# Autodesk Inventor assembly: ChalkBot_MasterAssem
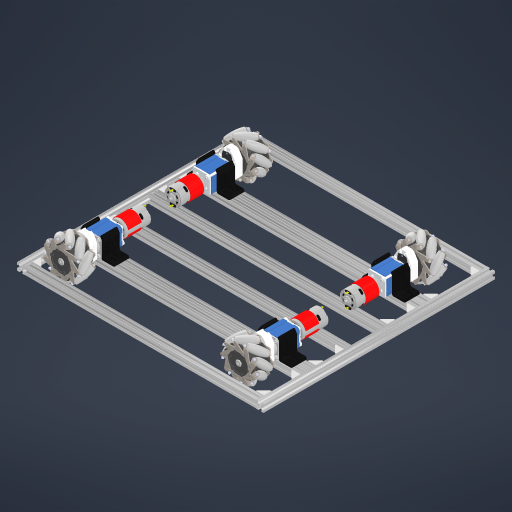
[picture p0: Inventor's stored thumbnail of the model, 512x512]
Saved by Autodesk Inventor 2024 (Build 280153000, 153)
## iProperties
Created: 2022-11-09
Part Number: ChalkBot_MasterAssem
Document SubType Name: Assembly
Designer: Dave
Author: Dave
## Documents named in this file (9)
- C:\Autodesk\ChalkBot Github\ChalkbotMechanical\Chalkbot1.0\ChalkBot_MasterAssem.iam
- C:\Users\Dave\Documents\GrabCAD\Chalk Bot\Chalkbot1.0\Chassis\V1\20x20 Channel.ipt
- C:\Autodesk\ChalkBot Github\ChalkbotMechanical\Chalkbot1.0\Chassis\V1\LeftMecanum-SubAssem01.iam
- C:\Autodesk\ChalkBot Github\ChalkbotMechanical\Chalkbot1.0\Chassis\V1\RightMecanum-SubAssem01.iam
- C:\Autodesk\ChalkBot Github\ChalkbotMechanical\Chalkbot1.0\Chassis\V1\20x20 90 Gusset.ipt
- C:\Autodesk\ChalkBot Github\ChalkbotMechanical\Chalkbot1.0\Chassis\V1\20x20 90 Gusset_MIR.ipt
- C:\Autodesk\ChalkBot Github\ChalkbotMechanical\Chalkbot1.0\Chassis\V1\20x20 90 Gusset_MIR1.ipt
- C:\Autodesk\ChalkBot Github\ChalkbotMechanical\Chalkbot1.0\Chassis\V1\20x20 90 Gusset_MIR_MIR.ipt
- C:\Autodesk\ChalkBot Github\ChalkbotMechanical\Chalkbot1.0\Chassis\V1\20x20 Channel\20x20 Channel-600.ipt
## Components (30 placed, 7 different names)
1. 20x20 Channel-600:1 — Flush:5, Flush:6, Flush:9, Flush:10, Mate:8, Flush:33, Mate:29, Tangent:7
2. 20x20 Channel-600:2 — Flush:6, Flush:7, Flush:8, Flush:9, Flush:27, Flush:28, Mate:4, Mate:5, Mate:6, Flush:32, Mate:28
3. 20x20 Channel-600:3 — Flush:7, Flush:8, Flush:15, Flush:16, Mate:12
4. 20x20 Channel-600:4 — Flush:2, Flush:3, Flush:12, Flush:13, Flush:17, Mate:16, Tangent:10
5. 20x20 Channel-600:5 — Flush:1, Flush:2, Flush:13, Flush:14, Mate:18, Tangent:9
6. 20x20 Channel-600:6 — Flush:1, Flush:14, Flush:29, Mate:20
7. 20x20 Channel-600:7 — Flush:3, Flush:4, Flush:11, Flush:12, Flush:16, Flush:17, Mate:15
8. 20x20 Channel-600:8 — Flush:4, Flush:5, Flush:10, Flush:11, Flush:15, Mate:11, Tangent:8
9. RightMecanum-SubAssem01:2 [sub-assembly] — Tangent:9, Tangent:10
10. LeftMecanum-SubAssem01:3 [sub-assembly]
11. RightMecanum-SubAssem01:1 [sub-assembly] — Flush:45
12. LeftMecanum-SubAssem01:4 [sub-assembly] — Tangent:7, Tangent:8, Flush:45
13. 20x20 Channel-600:9 — Flush:27, Flush:28, Mate:4, Flush:29, Flush:30, Flush:31, Mate:7, Mate:9, Flush:34, Mate:10, Mate:13, Flush:35, Mate:14, Mate:17, Mate:19, Mate:21
14. 20x20 Channel-600:10 — Flush:30, Flush:31, Mate:5, Mate:27, Flush:44
15. 20x20 90 Gusset:3 — Flush:34, Mate:10, Mate:11
16. 20x20 90 Gusset:4 — Mate:12, Mate:13, Flush:35, Flush:39
17. 20x20 90 Gusset:6 — Mate:6, Flush:32, Mate:7
18. 20x20 90 Gusset:7 — Mate:8, Mate:9, Flush:33
19. 20x20 90 Gusset_MIR:1 — Flush:36, Flush:37, Mate:16, Mate:17
20. 20x20 90 Gusset_MIR:2 — Flush:36, Flush:39, Mate:14, Mate:15
21. 20x20 90 Gusset_MIR:3 — Flush:38, Mate:20, Mate:21
22. 20x20 90 Gusset_MIR:4 — Flush:37, Flush:38, Mate:18, Mate:19
23. 20x20 90 Gusset_MIR1:1
24. 20x20 90 Gusset_MIR1:2 — Flush:40
25. 20x20 90 Gusset_MIR1:3 — Mate:27, Mate:28, Flush:44
26. 20x20 90 Gusset_MIR1:4 — Mate:29
27. 20x20 90 Gusset_MIR_MIR:1 — Flush:41, Flush:43
28. 20x20 90 Gusset_MIR_MIR:2 — Flush:40, Flush:41
29. 20x20 90 Gusset_MIR_MIR:3 — Flush:42
30. 20x20 90 Gusset_MIR_MIR:4 — Flush:42, Flush:43
## Relationships (70: Flush 41, Mate 22, Tangent 6, Symmetry 1)
- Flush:1: 20x20 Channel-600:5 ↔ 20x20 Channel-600:6
- Flush:2: 20x20 Channel-600:4 ↔ 20x20 Channel-600:5
- Flush:3: 20x20 Channel-600:4 ↔ 20x20 Channel-600:7
- Flush:4: 20x20 Channel-600:7 ↔ 20x20 Channel-600:8
- Flush:5: 20x20 Channel-600:1 ↔ 20x20 Channel-600:8
- Flush:6: 20x20 Channel-600:1 ↔ 20x20 Channel-600:2
- Flush:7: 20x20 Channel-600:2 ↔ 20x20 Channel-600:3
- Flush:8: 20x20 Channel-600:2 ↔ 20x20 Channel-600:3
- Flush:9: 20x20 Channel-600:1 ↔ 20x20 Channel-600:2
- Flush:10: 20x20 Channel-600:1 ↔ 20x20 Channel-600:8
- Flush:11: 20x20 Channel-600:7 ↔ 20x20 Channel-600:8
- Flush:12: 20x20 Channel-600:4 ↔ 20x20 Channel-600:7
- Flush:13: 20x20 Channel-600:4 ↔ 20x20 Channel-600:5
- Flush:14: 20x20 Channel-600:5 ↔ 20x20 Channel-600:6
- Flush:15 (93 mm): 20x20 Channel-600:3 ↔ 20x20 Channel-600:8
- Flush:16 (93 mm): 20x20 Channel-600:3 ↔ 20x20 Channel-600:7
- Flush:17 (93 mm): 20x20 Channel-600:4 ↔ 20x20 Channel-600:7
- [Flush]: RightMecanum-SubAssem01:1 ↔ LeftMecanum-SubAssem01:4
- [Flush]: RightMecanum-SubAssem01:2 ↔ LeftMecanum-SubAssem01:4
- [Flush]: RightMecanum-SubAssem01:2 ↔ LeftMecanum-SubAssem01:3
- [Mate]: 20x20 Channel-600:2 ↔ LeftMecanum-SubAssem01:4
- [Tangent] (1.0795 mm): 20x20 Channel-600:1 ↔ RightMecanum-SubAssem01:1
- [Tangent] (1.0795 mm): 20x20 Channel-600:5 ↔ LeftMecanum-SubAssem01:3
- [Flush]: LeftMecanum-SubAssem01:3 ↔ RightMecanum-SubAssem01:1
- [Flush]: RightMecanum-SubAssem01:2 ↔ LeftMecanum-SubAssem01:4
- [Symmetry]: RightMecanum-SubAssem01:1 ↔ LeftMecanum-SubAssem01:4
- Flush:27: 20x20 Channel-600:2 ↔ 20x20 Channel-600:9
- Flush:28: 20x20 Channel-600:2 ↔ 20x20 Channel-600:9
- Mate:4: 20x20 Channel-600:2 ↔ 20x20 Channel-600:9
- Flush:29: 20x20 Channel-600:6 ↔ 20x20 Channel-600:9
- Flush:30: 20x20 Channel-600:9 ↔ 20x20 Channel-600:10
- Flush:31: 20x20 Channel-600:9 ↔ 20x20 Channel-600:10
- Mate:5: 20x20 Channel-600:2 ↔ 20x20 Channel-600:10
- Mate:6: 20x20 Channel-600:2 ↔ 20x20 90 Gusset:6
- Flush:32: 20x20 Channel-600:2 ↔ 20x20 90 Gusset:6
- Mate:7: 20x20 Channel-600:9 ↔ 20x20 90 Gusset:6
- Mate:8: 20x20 Channel-600:1 ↔ 20x20 90 Gusset:7
- Mate:9: 20x20 Channel-600:9 ↔ 20x20 90 Gusset:7
- Flush:33: 20x20 Channel-600:1 ↔ 20x20 90 Gusset:7
- Flush:34: 20x20 Channel-600:9 ↔ 20x20 90 Gusset:3
- Mate:10: 20x20 Channel-600:9 ↔ 20x20 90 Gusset:3
- Mate:11: 20x20 Channel-600:8 ↔ 20x20 90 Gusset:3
- Mate:12: 20x20 Channel-600:3 ↔ 20x20 90 Gusset:4
- Mate:13: 20x20 Channel-600:9 ↔ 20x20 90 Gusset:4
- Flush:35: 20x20 Channel-600:9 ↔ 20x20 90 Gusset:4
- Flush:36: 20x20 90 Gusset_MIR:1 ↔ 20x20 90 Gusset_MIR:2
- Flush:37: 20x20 90 Gusset_MIR:1 ↔ 20x20 90 Gusset_MIR:4
- Flush:38: 20x20 90 Gusset_MIR:3 ↔ 20x20 90 Gusset_MIR:4
- Flush:39: 20x20 90 Gusset:4 ↔ 20x20 90 Gusset_MIR:2
- Mate:14: 20x20 Channel-600:9 ↔ 20x20 90 Gusset_MIR:2
- Mate:15: 20x20 Channel-600:7 ↔ 20x20 90 Gusset_MIR:2
- Mate:16: 20x20 Channel-600:4 ↔ 20x20 90 Gusset_MIR:1
- Mate:17: 20x20 Channel-600:9 ↔ 20x20 90 Gusset_MIR:1
- Mate:18: 20x20 Channel-600:5 ↔ 20x20 90 Gusset_MIR:4
- Mate:19: 20x20 Channel-600:9 ↔ 20x20 90 Gusset_MIR:4
- Mate:20: 20x20 Channel-600:6 ↔ 20x20 90 Gusset_MIR:3
- Mate:21: 20x20 Channel-600:9 ↔ 20x20 90 Gusset_MIR:3
- Flush:40: 20x20 90 Gusset_MIR1:2 ↔ 20x20 90 Gusset_MIR_MIR:2
- Flush:41: 20x20 90 Gusset_MIR_MIR:1 ↔ 20x20 90 Gusset_MIR_MIR:2
- Flush:42: 20x20 90 Gusset_MIR_MIR:3 ↔ 20x20 90 Gusset_MIR_MIR:4
- Flush:43: 20x20 90 Gusset_MIR_MIR:1 ↔ 20x20 90 Gusset_MIR_MIR:4
- Mate:27: 20x20 Channel-600:10 ↔ 20x20 90 Gusset_MIR1:3
- Mate:28: 20x20 Channel-600:2 ↔ 20x20 90 Gusset_MIR1:3
- Flush:44: 20x20 Channel-600:10 ↔ 20x20 90 Gusset_MIR1:3
- Mate:29: 20x20 Channel-600:1 ↔ 20x20 90 Gusset_MIR1:4
- Tangent:7: 20x20 Channel-600:1 ↔ LeftMecanum-SubAssem01:4
- Tangent:8: 20x20 Channel-600:8 ↔ LeftMecanum-SubAssem01:4
- Tangent:9: 20x20 Channel-600:5 ↔ RightMecanum-SubAssem01:2
- Tangent:10: 20x20 Channel-600:4 ↔ RightMecanum-SubAssem01:2
- Flush:45 (457.7334 mm): RightMecanum-SubAssem01:1 ↔ LeftMecanum-SubAssem01:4
